# Autodesk Inventor assembly: 振動ナイフモデル
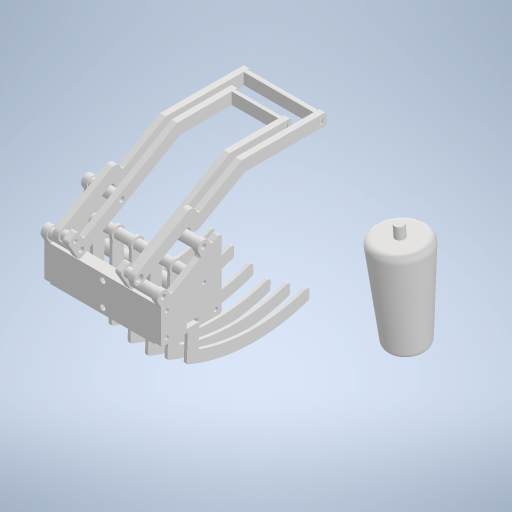
[picture p0: Inventor's stored thumbnail of the model, 512x512]
Saved by Autodesk Inventor 2024.3 (Build 283343000, 343)
## iProperties
Created: 2024-10-09
Part Number: 振動ナイフモデル
Document SubType Name: Assembly
Designer: hikou
Author: hikou
## Documents named in this file (17)
- C:\Users\hikou\OneDrive\ドキュメント\Inventor\end_effector\harvesting_endeffector\Vibrating_knife_endeffector\model\vibrating_knife_model.iam
- C:\Users\hikou\OneDrive\ドキュメント\Inventor\end_effector\harvesting_endeffector\Vibrating_knife_endeffector\model\stem_part.ipt
- C:\Users\hikou\OneDrive\ドキュメント\Inventor\end_effector\harvesting_endeffector\Vibrating_knife_endeffector\model\stem_part_atachment.ipt
- C:\Users\hikou\OneDrive\ドキュメント\Inventor\end_effector\harvesting_endeffector\Vibrating_knife_endeffector\model\base_part.ipt
- C:\Users\hikou\OneDrive\ドキュメント\Inventor\end_effector\harvesting_endeffector\Vibrating_knife_endeffector\model\base_part_finger.ipt
- C:\Users\hikou\OneDrive\ドキュメント\Inventor\end_effector\harvesting_endeffector\Vibrating_knife_endeffector\model\base_part_attachment.ipt
- C:\Users\hikou\OneDrive\ドキュメント\Inventor\end_effector\harvesting_endeffector\Vibrating_knife_endeffector\model\knife_attachment.ipt
- C:\Users\hikou\OneDrive\ドキュメント\Inventor\end_effector\harvesting_endeffector\Vibrating_knife_endeffector\model\knife_model.ipt
- C:\Users\hikou\OneDrive\ドキュメント\Inventor\end_effector\harvesting_endeffector\Vibrating_knife_endeffector\model\spacer4.4mm_in3.5mm.ipt
- C:\Users\hikou\OneDrive\ドキュメント\Inventor\end_effector\harvesting_endeffector\Vibrating_knife_endeffector\model\bearing_3mm.ipt
- C:\Users\hikou\OneDrive\ドキュメント\Inventor\end_effector\harvesting_endeffector\Vibrating_knife_endeffector\model\finger_L.ipt
- C:\Users\hikou\OneDrive\ドキュメント\Inventor\end_effector\harvesting_endeffector\Vibrating_knife_endeffector\model\spacer14mm_in3.5mm.ipt
- C:\Users\hikou\OneDrive\ドキュメント\Inventor\end_effector\harvesting_endeffector\Vibrating_knife_endeffector\model\finger_M.ipt
- C:\Users\hikou\OneDrive\ドキュメント\Inventor\end_effector\harvesting_endeffector\Vibrating_knife_endeffector\model\finger_S.ipt
- C:\Users\hikou\OneDrive\ドキュメント\Inventor\end_effector\harvesting_endeffector\Vibrating_knife_endeffector\model\green_pepper_model.ipt
- C:\Users\hikou\OneDrive\ドキュメント\Inventor\end_effector\harvesting_endeffector\Vibrating_knife_endeffector\model\spacer20mm_in4.3mm.ipt
- C:\Users\hikou\OneDrive\ドキュメント\Inventor\end_effector\harvesting_endeffector\Vibrating_knife_endeffector\model\spacer2.5mm_in3.3mm.ipt
## Components (38 placed, 16 different names)
1. stem_part:1 — メイト:4, メイト:5, メイト:6, 挿入:13
2. stem_part:2 — メイト:1, メイト:2, メイト:3, 挿入:12
3. stem_part_atachment:1 — メイト:1, メイト:2, メイト:3, メイト:4, メイト:5, メイト:6
4. base_part:1 — 挿入:1, 挿入:36, 挿入:43, 挿入:44, 挿入:48, 挿入:49
5. base_part:2 — 挿入:2, 挿入:4, 挿入:5, 挿入:37, 挿入:38, 挿入:46
6. base_part_finger:1 — 挿入:1, 挿入:2, 挿入:5
7. base_part_attachment:1 — 挿入:4, メイト:7, 挿入:36, 挿入:49
8. knife_attachment:1 — メイト:8, メイト:9, メイト:10, 挿入:41, 挿入:42
9. knife_attachment:2 — メイト:11, メイト:12, メイト:13, 挿入:16, 挿入:39, 挿入:40
10. knife_model:1 — メイト:8, メイト:9, メイト:10, メイト:11, メイト:12, メイト:13
11. spacer4.4mm_in3.5mm:1 — 挿入:15, 挿入:16
12. spacer4.4mm_in3.5mm:2 — 挿入:14
13. bearing_3mm:1 — 挿入:12, 挿入:15
14. bearing_3mm:2 — 挿入:13, 挿入:14
15. finger_L:1 — 挿入:17
16. finger_L:2 — 挿入:18
17. bearing_3mm:3 — 挿入:23, 挿入:25, 挿入:27
18. bearing_3mm:4 — 挿入:24, 挿入:26, 挿入:28
19. bearing_3mm:5 — 挿入:29, 挿入:31, 挿入:47
20. bearing_3mm:6 — 挿入:18, 挿入:20, 挿入:22
21. bearing_3mm:7 — 挿入:17, 挿入:19, 挿入:21
22. bearing_3mm:8 — 挿入:30, 挿入:32, 挿入:45
23. spacer14mm_in3.5mm:1 — 挿入:27, 挿入:31
24. spacer14mm_in3.5mm:2 — 挿入:28, 挿入:32
25. spacer14mm_in3.5mm:3 — 挿入:21, 挿入:25
26. spacer14mm_in3.5mm:4 — 挿入:22, 挿入:26
27. spacer14mm_in3.5mm:5 — 挿入:19, 挿入:20
28. finger_M:1 — 挿入:23
29. finger_M:2 — 挿入:24
30. finger_S:1 — 挿入:29
31. finger_S:2 — 挿入:30
32. green_pepper_model:1
33. spacer20mm_in4.3mm:1 — 挿入:41, 挿入:44
34. spacer20mm_in4.3mm:2 — 挿入:42, 挿入:43
35. spacer20mm_in4.3mm:3 — 挿入:38, 挿入:40
36. spacer20mm_in4.3mm:4 — 挿入:37, 挿入:39
37. spacer2.5mm_in3.3mm:1 — 挿入:47, 挿入:48
38. spacer2.5mm_in3.3mm:2 — 挿入:45, 挿入:46
## Relationships (52: Insert 39, Mate 13)
- メイト:1 [Mate]: stem_part:2 ↔ stem_part_atachment:1
- メイト:2 [Mate]: stem_part:2 ↔ stem_part_atachment:1
- メイト:3 [Mate]: stem_part:2 ↔ stem_part_atachment:1
- メイト:4 [Mate]: stem_part:1 ↔ stem_part_atachment:1
- メイト:5 [Mate]: stem_part:1 ↔ stem_part_atachment:1
- メイト:6 [Mate]: stem_part:1 ↔ stem_part_atachment:1
- 挿入:1 [Insert]: base_part:1 ↔ base_part_finger:1
- 挿入:2 [Insert]: base_part:2 ↔ base_part_finger:1
- 挿入:4 [Insert]: base_part:2 ↔ base_part_attachment:1
- メイト:7 [Mate]: base_part_attachment:1
- 挿入:5 [Insert]: base_part:2 ↔ base_part_finger:1
- メイト:8 [Mate]: knife_attachment:1 ↔ knife_model:1
- メイト:9 [Mate]: knife_attachment:1 ↔ knife_model:1
- メイト:10 [Mate]: knife_attachment:1 ↔ knife_model:1
- メイト:11 [Mate]: knife_attachment:2 ↔ knife_model:1
- メイト:12 [Mate]: knife_attachment:2 ↔ knife_model:1
- メイト:13 [Mate]: knife_attachment:2 ↔ knife_model:1
- 挿入:12 [Insert]: stem_part:2 ↔ bearing_3mm:1
- 挿入:13 [Insert]: stem_part:1 ↔ bearing_3mm:2
- 挿入:14 [Insert]: spacer4.4mm_in3.5mm:2 ↔ bearing_3mm:2
- 挿入:15 [Insert]: spacer4.4mm_in3.5mm:1 ↔ bearing_3mm:1
- 挿入:16 [Insert]: knife_attachment:2 ↔ spacer4.4mm_in3.5mm:1
- 挿入:17 [Insert]: finger_L:1 ↔ bearing_3mm:7
- 挿入:18 [Insert]: finger_L:2 ↔ bearing_3mm:6
- 挿入:19 [Insert]: bearing_3mm:7 ↔ spacer14mm_in3.5mm:5
- 挿入:20 [Insert]: bearing_3mm:6 ↔ spacer14mm_in3.5mm:5
- 挿入:21 [Insert]: bearing_3mm:7 ↔ spacer14mm_in3.5mm:3
- 挿入:22 [Insert]: bearing_3mm:6 ↔ spacer14mm_in3.5mm:4
- 挿入:23 [Insert]: bearing_3mm:3 ↔ finger_M:1
- 挿入:24 [Insert]: bearing_3mm:4 ↔ finger_M:2
- 挿入:25 [Insert]: bearing_3mm:3 ↔ spacer14mm_in3.5mm:3
- 挿入:26 [Insert]: bearing_3mm:4 ↔ spacer14mm_in3.5mm:4
- 挿入:27 [Insert]: bearing_3mm:3 ↔ spacer14mm_in3.5mm:1
- 挿入:28 [Insert]: bearing_3mm:4 ↔ spacer14mm_in3.5mm:2
- 挿入:29 [Insert]: bearing_3mm:5 ↔ finger_S:1
- 挿入:30 [Insert]: bearing_3mm:8 ↔ finger_S:2
- 挿入:31 [Insert]: bearing_3mm:5 ↔ spacer14mm_in3.5mm:1
- 挿入:32 [Insert]: bearing_3mm:8 ↔ spacer14mm_in3.5mm:2
- 挿入:36 [Insert]: base_part:1 ↔ base_part_attachment:1
- 挿入:37 [Insert]: base_part:2 ↔ spacer20mm_in4.3mm:4
- 挿入:38 [Insert]: base_part:2 ↔ spacer20mm_in4.3mm:3
- 挿入:39 [Insert]: knife_attachment:2 ↔ spacer20mm_in4.3mm:4
- 挿入:40 [Insert]: knife_attachment:2 ↔ spacer20mm_in4.3mm:3
- 挿入:41 [Insert]: knife_attachment:1 ↔ spacer20mm_in4.3mm:1
- 挿入:42 [Insert]: knife_attachment:1 ↔ spacer20mm_in4.3mm:2
- 挿入:43 [Insert]: base_part:1 ↔ spacer20mm_in4.3mm:2
- 挿入:44 [Insert]: base_part:1 ↔ spacer20mm_in4.3mm:1
- 挿入:45 [Insert]: bearing_3mm:8 ↔ spacer2.5mm_in3.3mm:2
- 挿入:46 [Insert]: base_part:2 ↔ spacer2.5mm_in3.3mm:2
- 挿入:47 [Insert]: bearing_3mm:5 ↔ spacer2.5mm_in3.3mm:1
- 挿入:48 [Insert]: base_part:1 ↔ spacer2.5mm_in3.3mm:1
- 挿入:49 [Insert]: base_part:1 ↔ base_part_attachment:1
